# Autodesk Inventor assembly: hat
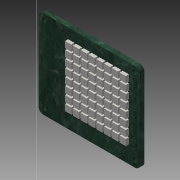
[picture p0: Inventor's stored thumbnail of the model, 180x180]
Saved by Autodesk Inventor 2015 (Build 190159000, 159)
## iProperties
Created: 2016-01-03
Part Number: hat
Document SubType Name: Assembly
Designer: david
Author: david
## Documents named in this file (4)
- Z:\gip\Inventor\generatie 7\Frame\Electronica\raspberry pi\hat.iam
- Z:\gip\Inventor\generatie 7\Frame\Electronica\raspberry pi\print.ipt
- Z:\gip\Inventor\generatie 7\Frame\Electronica\raspberry pi\LED.ipt
- Z:\gip\Inventor\generatie 7\Frame\Electronica\raspberry pi\GPIO_conector.ipt
## Components (66 placed, 3 different names)
1. print:1 — Mate:1, Flush:1, Flush:2
2. GPIO_conector:1
3. LED:1 — Mate:1, Flush:1, Flush:2
4. LED:2
5. LED:3
6. LED:4
7. LED:5
8. LED:6
9. LED:7
10. LED:8
11. LED:9
12. LED:10
13. LED:11
14. LED:12
15. LED:13
16. LED:14
17. LED:15
18. LED:16
19. LED:17
20. LED:18
21. LED:19
22. LED:20
23. LED:21
24. LED:22
25. LED:23
26. LED:24
27. LED:25
28. LED:26
29. LED:27
30. LED:28
31. LED:29
32. LED:30
33. LED:31
34. LED:32
35. LED:33
36. LED:34
37. LED:35
38. LED:36
39. LED:37
40. LED:38
41. LED:39
42. LED:40
43. LED:41
44. LED:42
45. LED:43
46. LED:44
47. LED:45
48. LED:46
49. LED:47
50. LED:48
51. LED:49
52. LED:50
53. LED:51
54. LED:52
55. LED:53
56. LED:54
57. LED:55
58. LED:56
59. LED:57
60. LED:58
61. LED:59
62. LED:60
63. LED:61
64. LED:62
65. LED:63
66. LED:64
## Component patterns: (64 elements, first: LED:1)
## Relationships (6: Flush 5, Mate 1)
- Mate:1: print:1 ↔ LED:1
- Flush:1 (11 mm): print:1 ↔ LED:1
- Flush:2 (-7 mm): print:1 ↔ LED:1
- [Flush] (-4 mm): print:1 ↔ GPIO_conector:1
- [Flush] (1 mm): print:1 ↔ GPIO_conector:1
- [Flush] (8 mm): print:1 ↔ GPIO_conector:1
